# Autodesk Inventor assembly: DeriveAssem
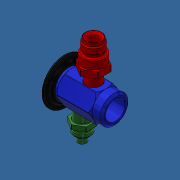
[picture p0: Inventor's stored thumbnail of the model, 180x180]
Saved by Autodesk Inventor 2022.4 (Build 264492010, 492A)
## iProperties
Created: 2009-04-14
Part Number: DeriveAssem
Document SubType Name: Assembly
Designer: User
Mass: 22.8734 g
Surface Area: 133.042 cm^2
Volume: 22.8734 cm^3
Density: 1 g/cm^3
CN_MASS: 0.02
Author: User
## Documents named in this file (5)
- U:\Inventor 2022 Training\_Designer Training\Inventor 2022 - Advanced Assembly\Practice Files\Derive Assem.iam
- U:\Inventor 2022 Training\_Designer Training\Inventor 2022 - Advanced Assembly\Practice Files\102650.ipt
- U:\Inventor 2022 Training\_Designer Training\Inventor 2022 - Advanced Assembly\Practice Files\102651.ipt
- U:\Inventor 2022 Training\_Designer Training\Inventor 2022 - Advanced Assembly\Practice Files\102652.ipt
- U:\Inventor 2022 Training\_Designer Training\Inventor 2022 - Advanced Assembly\Practice Files\102653.ipt
## Components (4 placed, 4 different names)
1. 102650:1 — Insert:1
2. 102652:2 — Insert:2
3. 102653:3 — Insert:1, Insert:2, Insert:3
4. 102651:4 — Insert:3
## Relationships (3: Insert 3)
- Insert:1: 102650:1 ↔ 102653:3
- Insert:2: 102652:2 ↔ 102653:3
- Insert:3: 102653:3 ↔ 102651:4
